# Autodesk Inventor assembly: Rev4StageSlider
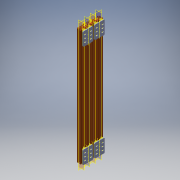
[picture p0: Inventor's stored thumbnail of the model, 180x180]
Saved by Autodesk Inventor 2018 (Build 220112000, 112)
## iProperties
Created: 2017-11-26
Part Number: Rev4StageSlider
Document SubType Name: Assembly
Designer: ball
Author: ball
## Documents named in this file (5)
- C:\FTC\FTC8863CAD\2017Robot\Rev4StageSlider.iam
- C:\FTC\FTC8863CAD\2017Robot\RevSingleStage.iam
- C:\FTC\FTC8863CAD\RevRobotics\REV-41-1039.ipt
- C:\FTC\FTC8863CAD\RevRobotics\REV-41-1094.ipt
- C:\FTC\FTC8863CAD\RevRobotics\REV-41-1095.ipt
## Components (16 placed, 4 different names)
1. RevSingleStage:1 [sub-assembly] — Mate:1, Flush:1, Mate:2, Flush:2, Flush:3, Flush:5, Mate:3, Flush:7, Flush:15, Flush:17, Flush:18, Mate:7, Flush:19, Flush:20, Mate:8, Flush:21, Flush:22, Flush:25, Flush:26, Mate:11, Flush:27, Mate:12, Mate:13
2. RevSingleStage:2 [sub-assembly] — Mate:1, Flush:1, Flush:6, Flush:15
3. REV-41-1039:1 — Mate:2, Flush:2, Flush:3, Flush:5
4. REV-41-1039:2 — Mate:3, Flush:6, Flush:7
5. RevSingleStage:8 [sub-assembly] — Flush:14
6. RevSingleStage:9 [sub-assembly] — Flush:14, Flush:21, Flush:22, Mate:9, Flush:23, Flush:24, Mate:10, Flush:28, Flush:29, Mate:14
7. REV-41-1039:3
8. REV-41-1039:4
9. REV-41-1094:2 — Flush:19, Flush:20, Mate:8, Mate:9, Flush:33
10. REV-41-1094:3 — Flush:17, Flush:18, Mate:7, Flush:31
11. REV-41-1095:5 — Flush:23, Flush:24, Mate:10, Mate:16
12. REV-41-1095:6 — Flush:28, Flush:29, Mate:14, Flush:30, Mate:15
13. REV-41-1095:7 — Flush:27, Mate:12, Mate:13
14. REV-41-1095:8 — Flush:25, Flush:26, Mate:11, Flush:32
15. REV-41-1039:5 — Flush:30, Flush:31, Mate:15
16. REV-41-1039:6 — Flush:32, Flush:33, Mate:16
## Relationships (47: Flush 31, Mate 16)
- Mate:1: RevSingleStage:1 ↔ RevSingleStage:2
- Flush:1: RevSingleStage:1 ↔ RevSingleStage:2
- Mate:2: RevSingleStage:1 ↔ REV-41-1039:1
- Flush:2: RevSingleStage:1 ↔ REV-41-1039:1
- Flush:3: RevSingleStage:1 ↔ REV-41-1039:1
- Flush:5: RevSingleStage:1 ↔ REV-41-1039:1
- Mate:3: RevSingleStage:1 ↔ REV-41-1039:2
- Flush:6: RevSingleStage:2 ↔ REV-41-1039:2
- Flush:7: RevSingleStage:1 ↔ REV-41-1039:2
- [Mate]: RevSingleStage:8 ↔ RevSingleStage:9
- [Flush]: RevSingleStage:8 ↔ RevSingleStage:9
- [Mate]: RevSingleStage:8 ↔ REV-41-1039:3
- [Flush]: RevSingleStage:8 ↔ REV-41-1039:3
- [Flush]: RevSingleStage:8 ↔ REV-41-1039:3
- [Flush]: RevSingleStage:8 ↔ REV-41-1039:3
- [Mate]: RevSingleStage:8 ↔ REV-41-1039:4
- [Flush]: RevSingleStage:9 ↔ REV-41-1039:4
- [Flush]: RevSingleStage:8 ↔ REV-41-1039:4
- Flush:14: RevSingleStage:8 ↔ RevSingleStage:9
- Flush:15: RevSingleStage:1 ↔ RevSingleStage:2
- Flush:17: RevSingleStage:1 ↔ REV-41-1094:3
- Flush:18: RevSingleStage:1 ↔ REV-41-1094:3
- Mate:7: RevSingleStage:1 ↔ REV-41-1094:3
- Flush:19: RevSingleStage:1 ↔ REV-41-1094:2
- Flush:20: RevSingleStage:1 ↔ REV-41-1094:2
- Mate:8: RevSingleStage:1 ↔ REV-41-1094:2
- Flush:21: RevSingleStage:1 ↔ RevSingleStage:9
- Flush:22: RevSingleStage:1 ↔ RevSingleStage:9
- Mate:9: RevSingleStage:9 ↔ REV-41-1094:2
- Flush:23: RevSingleStage:9 ↔ REV-41-1095:5
- Flush:24: RevSingleStage:9 ↔ REV-41-1095:5
- Mate:10: RevSingleStage:9 ↔ REV-41-1095:5
- Flush:25: RevSingleStage:1 ↔ REV-41-1095:8
- Flush:26: RevSingleStage:1 ↔ REV-41-1095:8
- Mate:11: RevSingleStage:1 ↔ REV-41-1095:8
- Flush:27: RevSingleStage:1 ↔ REV-41-1095:7
- Flush:28: RevSingleStage:9 ↔ REV-41-1095:6
- Mate:12: RevSingleStage:1 ↔ REV-41-1095:7
- Mate:13: RevSingleStage:1 ↔ REV-41-1095:7
- Flush:29: RevSingleStage:9 ↔ REV-41-1095:6
- Mate:14: RevSingleStage:9 ↔ REV-41-1095:6
- Flush:30: REV-41-1095:6 ↔ REV-41-1039:5
- Flush:31: REV-41-1094:3 ↔ REV-41-1039:5
- Mate:15: REV-41-1095:6 ↔ REV-41-1039:5
- Flush:32: REV-41-1095:8 ↔ REV-41-1039:6
- Flush:33: REV-41-1094:2 ↔ REV-41-1039:6
- Mate:16: REV-41-1095:5 ↔ REV-41-1039:6
## Named parameters: d12_d1 = 0 mm, d13_d2 = 0 mm, d14_d3 = 0 mm, d15_d4 = 0 mm, d16_d5 = 0 mm, d17_d8 = 0 mm, d18_d9 = 0 mm, d19_d10 = 0 mm, d20_d11 = 0 mm
